# Autodesk Inventor assembly: Assembly2
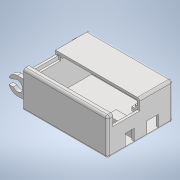
[picture p0: Inventor's stored thumbnail of the model, 180x180]
Saved by Autodesk Inventor 2020 (Build 240168000, 168)
## iProperties
Created: 2019-10-01
Part Number: Assembly2
Document SubType Name: Assembly
Designer: bzs3334
Mass: 117.324 g
Surface Area: 696.089 cm^2
Volume: 117.324 cm^3
Density: 1 g/cm^3
Author: bzs3334
## Documents named in this file (3)
- P:\LaserGazer\Assembly2.iam
- P:\LaserGazer\Case2.ipt
- P:\LaserGazer\Lid2.ipt
## Components (2 placed, 2 different names)
1. Case2:1 — Mate:1, Mate:2, Mate:3, Mate:5, Flush:1
2. Lid2:1 — Mate:5, Flush:1
## Relationships (5: Mate 4, Flush 1)
- Mate:1: Case2:1
- Mate:2: Case2:1
- Mate:3: Case2:1
- Mate:5: Case2:1 ↔ Lid2:1
- Flush:1: Case2:1 ↔ Lid2:1
